# Autodesk Inventor assembly: totaal_auto_v2
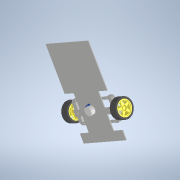
[picture p0: Inventor's stored thumbnail of the model, 180x180]
Saved by Autodesk Inventor 2022 (Build 260153000, 153)
## iProperties
Created: 2021-12-08
Part Number: totaal_auto_v2
Document SubType Name: Assembly
Designer: keemi
Author: keemi
## Documents named in this file (10)
- C:\Users\keemi\OneDrive\Documents\Inventor\Auto\totaal_auto_v2.iam
- C:\Users\keemi\OneDrive\Documents\Inventor\Auto\onderplaat v2.ipt
- C:\Users\keemi\OneDrive\Documents\Inventor\Auto\draaiarm voorwielen.ipt
- C:\Users\keemi\OneDrive\Documents\Inventor\Auto\stuur_arm v2.ipt
- C:\Users\keemi\OneDrive\Documents\Inventor\Auto\wheel-arduino-1.snapshot.2\Wheel ALL.ipt
- C:\Users\keemi\OneDrive\Documents\Inventor\Auto\staafje.ipt
- C:\Users\keemi\OneDrive\Documents\Inventor\Auto\tussenstaaf.ipt
- C:\Users\keemi\OneDrive\Documents\Inventor\Auto\Step - 28BYJ-48.ipt
- C:\Users\keemi\OneDrive\Documents\Inventor\Auto\stuurarm motor.ipt
- C:\Users\keemi\OneDrive\Documents\Inventor\Auto\tussenarmen_sturen.ipt
## Components (16 placed, 9 different names)
1. onderplaat v2:1 — Mate:6, Mate:7, Mate:8, Mate:9, Mate:18, Mate:32
2. draaiarm voorwielen:2 — Mate:1, Mate:2, Mate:3, Mate:4, Mate:5
3. stuur_arm v2:1 — Mate:4, Mate:5, Mate:15, Flush:2, Mate:27, Mate:29, Mate:31
4. Wheel ALL:1 — Mate:1, Mate:2, Mate:3
5. staafje:1 — Mate:6, Mate:7, Mate:15, Flush:2
6. staafje:2 — Mate:8, Mate:9, Mate:16, Flush:1
7. draaiarm voorwielen:3
8. stuur_arm v2:2 — Mate:16, Flush:1, Mate:28, Mate:30
9. Wheel ALL:2
10. tussenstaaf:1
11. Step - 28BYJ-48:1 — Mate:18, Mate:32
12. stuurarm motor:1 — Mate:19, Mate:21, Mate:23, Mate:24, Mate:25, Mate:26
13. tussenarmen_sturen:1 — Mate:19, Mate:20, Mate:26, Mate:29, Mate:31
14. tussenarmen_sturen:2 — Mate:21, Mate:22, Mate:24, Mate:27
15. tussenarmen_sturen:3 — Mate:22, Mate:23, Mate:28
16. tussenarmen_sturen:4 — Mate:20, Mate:25, Mate:30
## Relationships (33: Mate 31, Flush 2)
- Mate:1: draaiarm voorwielen:2 ↔ Wheel ALL:1
- Mate:2: draaiarm voorwielen:2 ↔ Wheel ALL:1
- Mate:3: draaiarm voorwielen:2 ↔ Wheel ALL:1
- Mate:4: draaiarm voorwielen:2 ↔ stuur_arm v2:1
- Mate:5: draaiarm voorwielen:2 ↔ stuur_arm v2:1
- Mate:6: onderplaat v2:1 ↔ staafje:1
- Mate:7: onderplaat v2:1 ↔ staafje:1
- Mate:8: onderplaat v2:1 ↔ staafje:2
- Mate:9: onderplaat v2:1 ↔ staafje:2
- [Mate]: draaiarm voorwielen:3 ↔ Wheel ALL:2
- [Mate]: draaiarm voorwielen:3 ↔ Wheel ALL:2
- [Mate]: draaiarm voorwielen:3 ↔ Wheel ALL:2
- [Mate]: draaiarm voorwielen:3 ↔ stuur_arm v2:2
- [Mate]: draaiarm voorwielen:3 ↔ stuur_arm v2:2
- Mate:15: stuur_arm v2:1 ↔ staafje:1
- Mate:16: staafje:2 ↔ stuur_arm v2:2
- Flush:1: staafje:2 ↔ stuur_arm v2:2
- Flush:2: stuur_arm v2:1 ↔ staafje:1
- Mate:18: onderplaat v2:1 ↔ Step - 28BYJ-48:1
- Mate:19: stuurarm motor:1 ↔ tussenarmen_sturen:1
- Mate:20: tussenarmen_sturen:1 ↔ tussenarmen_sturen:4
- Mate:21: stuurarm motor:1 ↔ tussenarmen_sturen:2
- Mate:22: tussenarmen_sturen:2 ↔ tussenarmen_sturen:3
- Mate:23: stuurarm motor:1 ↔ tussenarmen_sturen:3
- Mate:24: stuurarm motor:1 ↔ tussenarmen_sturen:2
- Mate:25: stuurarm motor:1 ↔ tussenarmen_sturen:4
- Mate:26: stuurarm motor:1 ↔ tussenarmen_sturen:1
- Mate:27: stuur_arm v2:1 ↔ tussenarmen_sturen:2
- Mate:28: stuur_arm v2:2 ↔ tussenarmen_sturen:3
- Mate:29: stuur_arm v2:1 ↔ tussenarmen_sturen:1
- Mate:30: stuur_arm v2:2 ↔ tussenarmen_sturen:4
- Mate:31: stuur_arm v2:1 ↔ tussenarmen_sturen:1
- Mate:32: onderplaat v2:1 ↔ Step - 28BYJ-48:1
## Named parameters: d12_d6 = 0 mm, d13_d7 = 0 mm, d14_d0 = 0 mm, d15_d1 = 0 mm, d16_d2 = 0 mm
